# Autodesk Inventor assembly: Cuerpo - Ensamble
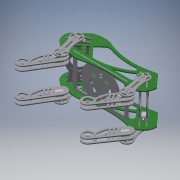
[picture p0: Inventor's stored thumbnail of the model, 180x180]
Saved by Autodesk Inventor 2019 (Build 230136000, 136)
## iProperties
Created: 2020-02-15
Part Number: Cuerpo - Ensamble
Material: Genérico
Document SubType Name: Assembly
Designer: Mafer1
Author: Mafer1
## Documents named in this file (8)
- E:\Escritorio\Temporal\Documentos\Robótica I\ProyectoCuadrupedo\Proyecto1\Proyecto1\Cuerpo - Ensamble.iam
- E:\Escritorio\Temporal\Documentos\Robótica I\ProyectoCuadrupedo\Proyecto1\Proyecto1\Cuerpo - Lateral.ipt
- E:\Escritorio\Temporal\Documentos\Robótica I\ProyectoCuadrupedo\Proyecto1\Proyecto1\Cuerpo - Base.ipt
- E:\Escritorio\Temporal\Documentos\Robótica I\ProyectoCuadrupedo\Proyecto1\Proyecto1\Cuerpo - Unión Laterales.ipt
- E:\Escritorio\Temporal\Documentos\Robótica I\ProyectoCuadrupedo\Proyecto1\Proyecto1\Pata - Ensamble.iam
- E:\Escritorio\Temporal\Documentos\Robótica I\ProyectoCuadrupedo\Proyecto1\Proyecto1\Pata - Ensamble_MIR.iam
- E:\Escritorio\Temporal\Documentos\Robótica I\ProyectoCuadrupedo\Proyecto1\Proyecto1\Pata - Ensamble Trasero.iam
- E:\Escritorio\Temporal\Documentos\Robótica I\ProyectoCuadrupedo\Proyecto1\Proyecto1\Pata - Ensamble Trasero_MIR.iam
## Components (11 placed, 7 different names)
1. Cuerpo - Lateral:2 — Coincidencia:1, Coincidencia:2, Coincidencia:3, Coincidencia:19, Coincidencia:20, Coincidencia:21, Coincidencia:31, Coincidencia:32, Coincidencia:33
2. Cuerpo - Base:1 — Coincidencia:1, Coincidencia:2, Coincidencia:3, Coincidencia:4, Coincidencia:5, Coincidencia:6
3. Cuerpo - Lateral:3 — Coincidencia:4, Coincidencia:5, Coincidencia:6, Coincidencia:7, Coincidencia:8, Coincidencia:9, Coincidencia:10, Coincidencia:11, Coincidencia:12, Coincidencia:13, Coincidencia:14, Coincidencia:15, Coincidencia:16, Coincidencia:17, Coincidencia:18, Coincidencia:22, Coincidencia:23, Coincidencia:24, Coincidencia:28, Coincidencia:29, Coincidencia:30
4. Cuerpo - Unión Laterales:1 — Coincidencia:7, Coincidencia:8, Coincidencia:9
5. Cuerpo - Unión Laterales:2 — Coincidencia:10, Coincidencia:11, Coincidencia:12
6. Cuerpo - Unión Laterales:3 — Coincidencia:13, Coincidencia:14, Coincidencia:15
7. Cuerpo - Unión Laterales:4 — Coincidencia:16, Coincidencia:17, Coincidencia:18
8. Pata - Ensamble:2 [sub-assembly] — Coincidencia:19, Coincidencia:20, Coincidencia:21
9. Pata - Ensamble_MIR:1 [sub-assembly] — Coincidencia:22, Coincidencia:23, Coincidencia:24
10. Pata - Ensamble Trasero_MIR:1 [sub-assembly] — Coincidencia:28, Coincidencia:29, Coincidencia:30
11. Pata - Ensamble Trasero:2 [sub-assembly] — Coincidencia:31, Coincidencia:32, Coincidencia:33
## Relationships (30: Mate 30)
- Coincidencia:1 [Mate] (-3.3 mm): Cuerpo - Lateral:2 ↔ Cuerpo - Base:1
- Coincidencia:2 [Mate]: Cuerpo - Lateral:2 ↔ Cuerpo - Base:1
- Coincidencia:3 [Mate]: Cuerpo - Lateral:2 ↔ Cuerpo - Base:1
- Coincidencia:4 [Mate] (-3.3 mm): Cuerpo - Base:1 ↔ Cuerpo - Lateral:3
- Coincidencia:5 [Mate]: Cuerpo - Base:1 ↔ Cuerpo - Lateral:3
- Coincidencia:6 [Mate]: Cuerpo - Base:1 ↔ Cuerpo - Lateral:3
- Coincidencia:7 [Mate]: Cuerpo - Lateral:3 ↔ Cuerpo - Unión Laterales:1
- Coincidencia:8 [Mate]: Cuerpo - Lateral:3 ↔ Cuerpo - Unión Laterales:1
- Coincidencia:9 [Mate]: Cuerpo - Lateral:3 ↔ Cuerpo - Unión Laterales:1
- Coincidencia:10 [Mate]: Cuerpo - Lateral:3 ↔ Cuerpo - Unión Laterales:2
- Coincidencia:11 [Mate]: Cuerpo - Lateral:3 ↔ Cuerpo - Unión Laterales:2
- Coincidencia:12 [Mate]: Cuerpo - Lateral:3 ↔ Cuerpo - Unión Laterales:2
- Coincidencia:13 [Mate]: Cuerpo - Lateral:3 ↔ Cuerpo - Unión Laterales:3
- Coincidencia:14 [Mate]: Cuerpo - Lateral:3 ↔ Cuerpo - Unión Laterales:3
- Coincidencia:15 [Mate]: Cuerpo - Lateral:3 ↔ Cuerpo - Unión Laterales:3
- Coincidencia:16 [Mate]: Cuerpo - Lateral:3 ↔ Cuerpo - Unión Laterales:4
- Coincidencia:17 [Mate]: Cuerpo - Lateral:3 ↔ Cuerpo - Unión Laterales:4
- Coincidencia:18 [Mate]: Cuerpo - Lateral:3 ↔ Cuerpo - Unión Laterales:4
- Coincidencia:19 [Mate]: Cuerpo - Lateral:2 ↔ Pata - Ensamble:2
- Coincidencia:20 [Mate]: Cuerpo - Lateral:2 ↔ Pata - Ensamble:2
- Coincidencia:21 [Mate]: Cuerpo - Lateral:2 ↔ Pata - Ensamble:2
- Coincidencia:22 [Mate]: Cuerpo - Lateral:3 ↔ Pata - Ensamble_MIR:1
- Coincidencia:23 [Mate]: Cuerpo - Lateral:3 ↔ Pata - Ensamble_MIR:1
- Coincidencia:24 [Mate]: Cuerpo - Lateral:3 ↔ Pata - Ensamble_MIR:1
- Coincidencia:28 [Mate]: Cuerpo - Lateral:3 ↔ Pata - Ensamble Trasero_MIR:1
- Coincidencia:29 [Mate]: Cuerpo - Lateral:3 ↔ Pata - Ensamble Trasero_MIR:1
- Coincidencia:30 [Mate]: Cuerpo - Lateral:3 ↔ Pata - Ensamble Trasero_MIR:1
- Coincidencia:31 [Mate]: Cuerpo - Lateral:2 ↔ Pata - Ensamble Trasero:2
- Coincidencia:32 [Mate]: Cuerpo - Lateral:2 ↔ Pata - Ensamble Trasero:2
- Coincidencia:33 [Mate]: Cuerpo - Lateral:2 ↔ Pata - Ensamble Trasero:2
